# Autodesk Inventor assembly: Assembly1
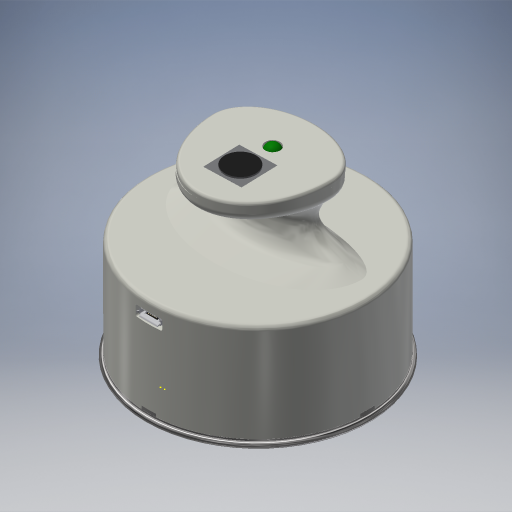
[picture p0: Inventor's stored thumbnail of the model, 512x512]
Saved by Autodesk Inventor 2023 (Build 270158000, 158)
## iProperties
Created: 2023-10-24
Part Number: Assembly1
Document SubType Name: Assembly
Designer: czair
Author: czair
## Documents named in this file (12)
- C:\Users\czair\Downloads\Assembly1.iam
- C:\Users\czair\Downloads\Boton.ipt
- C:\Users\czair\Downloads\Tapa.ipt
- C:\Users\czair\Downloads\Placa.ipt
- C:\Users\czair\Downloads\Carcasa.ipt
- C:\Users\czair\Downloads\BTG_901_BT_003_LED_5mm_Green\LED_5mm_Green.ipt
- C:\Users\czair\Downloads\Nano33BLE\Nano33BLE.ipt
- C:\Users\czair\Downloads\TP4056 .ipt
- C:\Users\czair\Downloads\micro-sd-card-module-step-1.snapshot.1\leitor microsd.ipt
- C:\Users\czair\Downloads\9x12-buzzer-1.snapshot.1\9x12 Buzzer.ipt
- C:\Users\czair\Downloads\bateria-lipo-3-7v-1000-ma-1.snapshot.1\Bateria LiPo 3.7V 1000mA 503450 v23.ipt
- C:\Users\czair\Downloads\microfone-de-eletreto-1.snapshot.2\microfone.ipt
## Components (11 placed, 11 different names)
1. Boton:1 — Mate:3, Mate:4, Flush:1
2. Tapa:1 — Mate:3, Mate:4, Flush:1, Mate:9, Mate:10, Mate:12, Mate:15
3. Placa:1 — Mate:13, Mate:14, Mate:16, Flush:2
4. LED_5mm_Green:1 — Mate:15
5. Nano33BLE:1
6. TP4056 :1 — Mate:5, Mate:6, Mate:8
7. leitor microsd:1
8. Carcasa:1 — Mate:5, Mate:6, Mate:8, Mate:9, Mate:10, Mate:12, Mate:13, Mate:14
9. 9x12 Buzzer:1
10. Bateria LiPo 3.7V 1000mA 503450 v23:1
11. microfone:1 — Mate:16, Flush:2
## Relationships (14: Mate 12, Flush 2)
- Mate:3: Boton:1 ↔ Tapa:1
- Mate:4: Boton:1 ↔ Tapa:1
- Flush:1: Boton:1 ↔ Tapa:1
- Mate:5: TP4056 :1 ↔ Carcasa:1
- Mate:6: TP4056 :1 ↔ Carcasa:1
- Mate:8: TP4056 :1 ↔ Carcasa:1
- Mate:9: Tapa:1 ↔ Carcasa:1
- Mate:10: Tapa:1 ↔ Carcasa:1
- Mate:12: Tapa:1 ↔ Carcasa:1
- Mate:13: Placa:1 ↔ Carcasa:1
- Mate:14: Placa:1 ↔ Carcasa:1
- Mate:15: Tapa:1 ↔ LED_5mm_Green:1
- Mate:16: Placa:1 ↔ microfone:1
- Flush:2: Placa:1 ↔ microfone:1
